# Autodesk Inventor assembly: legAssemblyV2
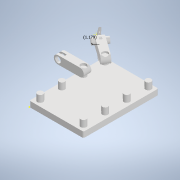
[picture p0: Inventor's stored thumbnail of the model, 180x180]
Saved by Autodesk Inventor 2022 (Build 260153000, 153)
## iProperties
Created: 2022-01-24
Part Number: legAssemblyV2
Document SubType Name: Assembly
Designer: money
Author: money
## Documents named in this file (5)
- C:\Users\money\Documents\Inventor\A2-Alternate-Mobility-Hand\legAssemblyV2.iam
- C:\Users\money\Documents\Inventor\A2-Alternate-Mobility-Hand\legV2.ipt
- C:\Users\money\Documents\Inventor\A2-Alternate-Mobility-Hand\toplegV2.ipt
- C:\Users\money\Documents\Inventor\A2-Alternate-Mobility-Hand\jointV0.ipt
- C:\Users\money\Documents\Inventor\A2-Alternate-Mobility-Hand\BasePlateV1.ipt
## Components (5 placed, 4 different names)
1. legV2:1 — Insert:3
2. toplegV2:1 — Insert:2, Insert:4
3. jointV0:1 — Insert:2, Insert:3
4. BasePlateV1:1 — Insert:4, Insert:5
5. toplegV2:2 — Insert:5
## Relationships (4: Insert 4)
- Insert:2 (-6.35 mm): toplegV2:1 ↔ jointV0:1
- Insert:3 (-19.05 mm): legV2:1 ↔ jointV0:1
- Insert:4 (3.81 mm): toplegV2:1 ↔ BasePlateV1:1
- Insert:5 (-5.08 mm): BasePlateV1:1 ↔ toplegV2:2
